# Autodesk Inventor assembly: ENSAMBLE MECANISMO DE INGRESO
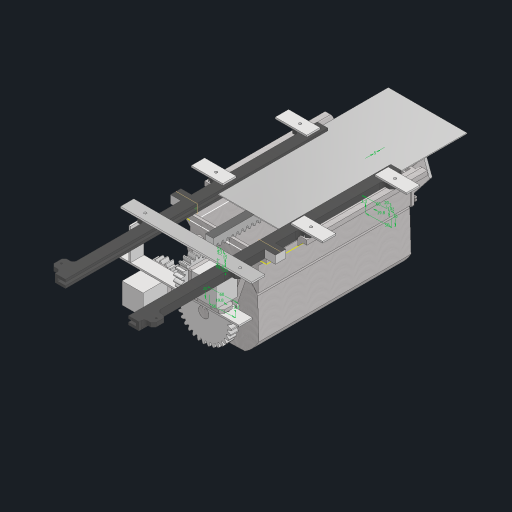
[picture p0: Inventor's stored thumbnail of the model, 512x512]
Saved by Autodesk Inventor 2024.3 (Build 283343000, 343)
## iProperties
Created: 2024-06-13
Part Number: ENSAMBLE MECANISMO DE INGRESO
Document SubType Name: Assembly
Designer: Jhuliams
Author: Jhuliams
## Documents named in this file (25)
- C:\Users\Niler\OneDrive\Escritorio\RECICLADOR\RECICLADOR_MODELO_3D\MECANISMO DE COMPACTADO\ENSAMBLE MECANISMO DE INGRESO.iam
- C:\Users\Niler\OneDrive\Escritorio\RECICLADOR\RECICLADOR_MODELO_3D\MECANISMO DE COMPACTADO\PINON DE TAPA PRINCIPAL.ipt
- C:\Users\Niler\OneDrive\Escritorio\RECICLADOR\RECICLADOR_MODELO_3D\MECANISMO DE COMPACTADO\TAPA PRICIPAL CON CREMALLERA.ipt
- C:\Users\Niler\OneDrive\Escritorio\RECICLADOR\RECICLADOR_MODELO_3D\MECANISMO DE COMPACTADO\GUIA DE TAPA PRINCIPAL.ipt
- C:\Users\Niler\OneDrive\Escritorio\RECICLADOR\RECICLADOR_MODELO_3D\MECANISMO DE COMPACTADO\NEMA 17 PARA TAPA PRINCIPAL.ipt
- C:\Users\Niler\OneDrive\Escritorio\RECICLADOR\RECICLADOR_MODELO_3D\MECANISMO DE COMPACTADO\PLETINA PARA CARA INCLINADA.ipt
- C:\Users\Niler\OneDrive\Escritorio\RECICLADOR\RECICLADOR_MODELO_3D\MECANISMO DE COMPACTADO\PLETINA PARA CARA INCLINADA_2.ipt
- C:\Users\Niler\OneDrive\Escritorio\RECICLADOR\RECICLADOR_MODELO_3D\MECANISMO DE COMPACTADO\ACOPLE_NEMA_PUERTA.ipt
- C:\Users\Niler\OneDrive\Escritorio\RECICLADOR\RECICLADOR_MODELO_3D\MECANISMO DE COMPACTADO\TOBOGAN_BASURA.ipt
- C:\Users\Niler\OneDrive\Escritorio\RECICLADOR\RECICLADOR_MODELO_3D\MECANISMO DE COMPACTADO\COMPUERTA_ALUMINIO.ipt
- C:\Users\Niler\OneDrive\Escritorio\RECICLADOR\RECICLADOR_MODELO_3D\MECANISMO DE COMPACTADO\PUERTA_ACOPLE_ENTRADA_v2.ipt
- C:\Users\Niler\OneDrive\Escritorio\RECICLADOR\RECICLADOR_MODELO_3D\MECANISMO DE COMPACTADO\CAJA_V2.ipt
- C:\Users\Niler\OneDrive\Escritorio\RECICLADOR\RECICLADOR_MODELO_3D\MECANISMO DE COMPACTADO\GIRO_1.ipt
- C:\Users\Niler\OneDrive\Escritorio\RECICLADOR\RECICLADOR_MODELO_3D\MECANISMO DE COMPACTADO\GIRO_2.ipt
- C:\Users\Niler\OneDrive\Escritorio\RECICLADOR\RECICLADOR_MODELO_3D\MECANISMO DE COMPACTADO\SOPORTE_RODAMIENTO.ipt
- C:\Users\Niler\OneDrive\Escritorio\RECICLADOR\RECICLADOR_MODELO_3D\MECANISMO DE COMPACTADO\ACOPLE_NEMA_PUERTA_V2.ipt
- C:\Users\Niler\OneDrive\Escritorio\RECICLADOR\RECICLADOR_MODELO_3D\MECANISMO DE COMPACTADO\ENGRANAJE CONDUCTOR DE CAJA.ipt
- C:\Users\Niler\OneDrive\Escritorio\RECICLADOR\RECICLADOR_MODELO_3D\MECANISMO DE COMPACTADO\ENGRANE MOTRIZ DE CAJA.ipt
- C:\Users\Niler\OneDrive\Escritorio\RECICLADOR\RECICLADOR_MODELO_3D\MECANISMO DE COMPACTADO\MUESCA_DETECCION_CERO.ipt
- C:\Users\Niler\OneDrive\Escritorio\RECICLADOR\RECICLADOR_MODELO_3D\VERSION_3_COMPLETA\CAMARA.ipt
- C:\Users\Niler\OneDrive\Escritorio\RECICLADOR\RECICLADOR_MODELO_3D\VERSION_3_COMPLETA\SOPORTE_CAMARA_2.ipt
- C:\Users\Niler\OneDrive\Escritorio\RECICLADOR\RECICLADOR_MODELO_3D\VERSION_3_COMPLETA\FIN_DE_CARRERA.ipt
- C:\Users\Niler\OneDrive\Escritorio\RECICLADOR\RECICLADOR_MODELO_3D\VERSION_3_COMPLETA\SOPORTE_FIN_CARRERA_INGRESO.ipt
- C:\Users\Niler\OneDrive\Escritorio\RECICLADOR\RECICLADOR_MODELO_3D\VERSION_3_COMPLETA\CIRCULAR_FIN_DE_CARRERA.ipt
- C:\Users\Niler\OneDrive\Escritorio\RECICLADOR\RECICLADOR_MODELO_3D\VERSION_3_COMPLETA\TAPA_CAMARA_2.ipt
## Components (34 placed, 24 different names)
1. PINON DE TAPA PRINCIPAL:1 — Mate:7, Mate:8, Mate:29, Flush:20, Rotation/Translation:1
2. NEMA 17 PARA TAPA PRINCIPAL:1 — Mate:7, Mate:8, Mate:30, Mate:31, Mate:32, Angle:1
3. PLETINA PARA CARA INCLINADA:1 — Flush:16, Flush:17, Mate:12, Mate:13, Mate:14, Mate:16, Mate:24, Mate:30, Mate:33, Flush:21
4. PLETINA PARA CARA INCLINADA_2:1 — Flush:16, Mate:18, Mate:23, Flush:19
5. PLETINA PARA CARA INCLINADA_2:2 — Flush:17, Mate:19, Mate:20, Flush:18
6. GUIA DE TAPA PRINCIPAL:3 — Mate:14, Mate:16, Mate:18, Mate:23, Mate:26, Mate:28, Angle:2, Symmetry:1
7. GUIA DE TAPA PRINCIPAL:4 — Mate:13, Mate:19, Mate:20, Mate:24, Mate:25, Mate:27, Angle:3, Mate:42, Symmetry:1
8. TAPA PRICIPAL CON CREMALLERA:1 — Mate:29, Flush:20, Rotation/Translation:1, Mate:38, Angle:3, Mate:44, Mate:45, Mate:89
9. PLETINA PARA CARA INCLINADA_2:3 — Mate:25, Flush:18, Mate:27, Mate:37, Mate:41
10. PLETINA PARA CARA INCLINADA_2:4 — Mate:26, Flush:19, Mate:28, Mate:36, Mate:40
11. ACOPLE_NEMA_PUERTA:1 — Mate:31, Mate:32, Angle:1, Angle:2, Mate:39
12. PLETINA PARA CARA INCLINADA_2:5 — Mate:33, Flush:21, Mate:34, Flush:22
13. PLETINA PARA CARA INCLINADA:2 — Mate:34, Flush:22, Mate:35, Flush:23, Mate:39, Mate:57, Flush:26
14. PLETINA PARA CARA INCLINADA_2:6 — Mate:35, Flush:23
15. TOBOGAN_BASURA:1 — Mate:36, Mate:37
16. COMPUERTA_ALUMINIO:1 — Mate:38, Mate:44, Mate:89
17. PUERTA_ACOPLE_ENTRADA_v2:1 — Mate:40, Mate:41, Mate:42, Flush:24, Mate:43, Mate:51, Mate:52, Mate:53, Mate:55, Mate:56, Mate:79, Mate:80, Mate:81
18. CAJA_V2:1 — Flush:24, Mate:43, Mate:46, Mate:48, Mate:49, Mate:50, Mate:54, Mate:66, Mate:67, Mate:68, Mate:69
19. GIRO_1:1 — Mate:46, Mate:48, Mate:61, Flush:28, Mate:69
20. GIRO_2:1 — Mate:49, Mate:50, Mate:85, Mate:86, Mate:87
21. SOPORTE_RODAMIENTO:1 — Mate:51, Mate:52, Mate:53, Mate:73, Mate:74, Mate:75
22. SOPORTE_RODAMIENTO:2 — Mate:54, Mate:55, Mate:56
23. ACOPLE_NEMA_PUERTA_V2:1 — Mate:57, Flush:26, Mate:59, Flush:27, Mate:60
24. ENGRANAJE CONDUCTOR DE CAJA:1 — Mate:61, Flush:28
25. ENGRANE MOTRIZ DE CAJA:1 — Mate:62
26. NEMA 17 PARA TAPA PRINCIPAL:2 — Mate:59, Flush:27, Mate:60, Mate:62
27. MUESCA_DETECCION_CERO:1 — Mate:66, Mate:67, Mate:68
28. SOPORTE_CAMARA_2:1 — Mate:70, Mate:73, Mate:74, Mate:75, Mate:76, Mate:77, Mate:78, Flush:29, Mate:88
29. CAMARA:1 — Mate:70
30. FIN_DE_CARRERA:1 — Mate:76, Mate:77, Mate:78
31. SOPORTE_FIN_CARRERA_INGRESO:1 — Mate:79, Mate:80, Mate:81, Mate:82, Mate:83, Mate:84
32. FIN_DE_CARRERA:2 — Mate:82, Mate:83, Mate:84
33. CIRCULAR_FIN_DE_CARRERA:1 — Mate:85, Mate:86, Mate:87
34. TAPA_CAMARA_2:1 — Flush:29, Mate:88
## Relationships (91: Mate 70, Flush 15, Angle 3, RelateRotateTranslate 1, Symmetry 1, RelateRotation 1)
- Flush:4 (27 mm)
- Mate:7: PINON DE TAPA PRINCIPAL:1 ↔ NEMA 17 PARA TAPA PRINCIPAL:1
- Mate:8 (10 mm): PINON DE TAPA PRINCIPAL:1 ↔ NEMA 17 PARA TAPA PRINCIPAL:1
- Flush:16: PLETINA PARA CARA INCLINADA:1 ↔ PLETINA PARA CARA INCLINADA_2:1
- Flush:17: PLETINA PARA CARA INCLINADA:1 ↔ PLETINA PARA CARA INCLINADA_2:2
- Mate:12: PLETINA PARA CARA INCLINADA:1
- Mate:13: PLETINA PARA CARA INCLINADA:1 ↔ GUIA DE TAPA PRINCIPAL:4
- Mate:14: PLETINA PARA CARA INCLINADA:1 ↔ GUIA DE TAPA PRINCIPAL:3
- Mate:16: PLETINA PARA CARA INCLINADA:1 ↔ GUIA DE TAPA PRINCIPAL:3
- Mate:18: PLETINA PARA CARA INCLINADA_2:1 ↔ GUIA DE TAPA PRINCIPAL:3
- Mate:19: PLETINA PARA CARA INCLINADA_2:2 ↔ GUIA DE TAPA PRINCIPAL:4
- Mate:20: PLETINA PARA CARA INCLINADA_2:2 ↔ GUIA DE TAPA PRINCIPAL:4
- Mate:23: PLETINA PARA CARA INCLINADA_2:1 ↔ GUIA DE TAPA PRINCIPAL:3
- Mate:24: PLETINA PARA CARA INCLINADA:1 ↔ GUIA DE TAPA PRINCIPAL:4
- Mate:25: GUIA DE TAPA PRINCIPAL:4 ↔ PLETINA PARA CARA INCLINADA_2:3
- Flush:18: PLETINA PARA CARA INCLINADA_2:2 ↔ PLETINA PARA CARA INCLINADA_2:3
- Mate:26: GUIA DE TAPA PRINCIPAL:3 ↔ PLETINA PARA CARA INCLINADA_2:4
- Flush:19: PLETINA PARA CARA INCLINADA_2:1 ↔ PLETINA PARA CARA INCLINADA_2:4
- Mate:27: GUIA DE TAPA PRINCIPAL:4 ↔ PLETINA PARA CARA INCLINADA_2:3
- Mate:28: GUIA DE TAPA PRINCIPAL:3 ↔ PLETINA PARA CARA INCLINADA_2:4
- Mate:29 (30.4 mm): PINON DE TAPA PRINCIPAL:1 ↔ TAPA PRICIPAL CON CREMALLERA:1
- Flush:20: PINON DE TAPA PRINCIPAL:1 ↔ TAPA PRICIPAL CON CREMALLERA:1
- Mate:30: NEMA 17 PARA TAPA PRINCIPAL:1 ↔ PLETINA PARA CARA INCLINADA:1
- Rotation/Translation:1 [RelateRotateTranslate] (169 mm): PINON DE TAPA PRINCIPAL:1 ↔ TAPA PRICIPAL CON CREMALLERA:1
- Mate:31: NEMA 17 PARA TAPA PRINCIPAL:1 ↔ ACOPLE_NEMA_PUERTA:1
- Mate:32: NEMA 17 PARA TAPA PRINCIPAL:1 ↔ ACOPLE_NEMA_PUERTA:1
- Angle:1 (0 deg): NEMA 17 PARA TAPA PRINCIPAL:1 ↔ ACOPLE_NEMA_PUERTA:1
- Angle:2 (0 deg): GUIA DE TAPA PRINCIPAL:3 ↔ ACOPLE_NEMA_PUERTA:1
- Mate:33 (20 mm): PLETINA PARA CARA INCLINADA:1 ↔ PLETINA PARA CARA INCLINADA_2:5
- Flush:21: PLETINA PARA CARA INCLINADA:1 ↔ PLETINA PARA CARA INCLINADA_2:5
- Mate:34: PLETINA PARA CARA INCLINADA_2:5 ↔ PLETINA PARA CARA INCLINADA:2
- Flush:22: PLETINA PARA CARA INCLINADA_2:5 ↔ PLETINA PARA CARA INCLINADA:2
- Mate:35: PLETINA PARA CARA INCLINADA:2 ↔ PLETINA PARA CARA INCLINADA_2:6
- Flush:23: PLETINA PARA CARA INCLINADA:2 ↔ PLETINA PARA CARA INCLINADA_2:6
- Mate:36: PLETINA PARA CARA INCLINADA_2:4 ↔ TOBOGAN_BASURA:1
- Mate:37: PLETINA PARA CARA INCLINADA_2:3 ↔ TOBOGAN_BASURA:1
- Mate:38: TAPA PRICIPAL CON CREMALLERA:1 ↔ COMPUERTA_ALUMINIO:1
- Mate:39: ACOPLE_NEMA_PUERTA:1 ↔ PLETINA PARA CARA INCLINADA:2
- Angle:3 (0 deg): GUIA DE TAPA PRINCIPAL:4 ↔ TAPA PRICIPAL CON CREMALLERA:1
- Mate:40: PLETINA PARA CARA INCLINADA_2:4 ↔ PUERTA_ACOPLE_ENTRADA_v2:1
- Mate:41: PLETINA PARA CARA INCLINADA_2:3 ↔ PUERTA_ACOPLE_ENTRADA_v2:1
- Mate:42: GUIA DE TAPA PRINCIPAL:4 ↔ PUERTA_ACOPLE_ENTRADA_v2:1
- Flush:24: PUERTA_ACOPLE_ENTRADA_v2:1 ↔ CAJA_V2:1
- Mate:43: PUERTA_ACOPLE_ENTRADA_v2:1 ↔ CAJA_V2:1
- Mate:44: TAPA PRICIPAL CON CREMALLERA:1 ↔ COMPUERTA_ALUMINIO:1
- Symmetry:1: GUIA DE TAPA PRINCIPAL:3 ↔ GUIA DE TAPA PRINCIPAL:4
- Mate:45: TAPA PRICIPAL CON CREMALLERA:1
- Mate:46: CAJA_V2:1 ↔ GIRO_1:1
- Mate:48: CAJA_V2:1 ↔ GIRO_1:1
- Mate:49: CAJA_V2:1 ↔ GIRO_2:1
- Mate:50: CAJA_V2:1 ↔ GIRO_2:1
- Mate:51: PUERTA_ACOPLE_ENTRADA_v2:1 ↔ SOPORTE_RODAMIENTO:1
- Mate:52: PUERTA_ACOPLE_ENTRADA_v2:1 ↔ SOPORTE_RODAMIENTO:1
- Mate:53: PUERTA_ACOPLE_ENTRADA_v2:1 ↔ SOPORTE_RODAMIENTO:1
- Mate:54: CAJA_V2:1 ↔ SOPORTE_RODAMIENTO:2
- Mate:55: PUERTA_ACOPLE_ENTRADA_v2:1 ↔ SOPORTE_RODAMIENTO:2
- Mate:56: PUERTA_ACOPLE_ENTRADA_v2:1 ↔ SOPORTE_RODAMIENTO:2
- Mate:57: PLETINA PARA CARA INCLINADA:2 ↔ ACOPLE_NEMA_PUERTA_V2:1
- [Flush]: ENGRANAJE CONDUCTOR DE CAJA:1 ↔ ENGRANE MOTRIZ DE CAJA:1
- [Mate] (79.5 mm): ENGRANAJE CONDUCTOR DE CAJA:1 ↔ ENGRANE MOTRIZ DE CAJA:1
- [RelateRotation] (1.65 ul): ENGRANAJE CONDUCTOR DE CAJA:1 ↔ ENGRANE MOTRIZ DE CAJA:1
- Flush:26 (-5 mm): PLETINA PARA CARA INCLINADA:2 ↔ ACOPLE_NEMA_PUERTA_V2:1
- Mate:59: ACOPLE_NEMA_PUERTA_V2:1 ↔ NEMA 17 PARA TAPA PRINCIPAL:2
- Flush:27: ACOPLE_NEMA_PUERTA_V2:1 ↔ NEMA 17 PARA TAPA PRINCIPAL:2
- Mate:60: ACOPLE_NEMA_PUERTA_V2:1 ↔ NEMA 17 PARA TAPA PRINCIPAL:2
- Mate:61: GIRO_1:1 ↔ ENGRANAJE CONDUCTOR DE CAJA:1
- Mate:62: ENGRANE MOTRIZ DE CAJA:1 ↔ NEMA 17 PARA TAPA PRINCIPAL:2
- Flush:28: GIRO_1:1 ↔ ENGRANAJE CONDUCTOR DE CAJA:1
- Mate:66: CAJA_V2:1 ↔ MUESCA_DETECCION_CERO:1
- Mate:67: CAJA_V2:1 ↔ MUESCA_DETECCION_CERO:1
- Mate:68: CAJA_V2:1 ↔ MUESCA_DETECCION_CERO:1
- Mate:69: CAJA_V2:1 ↔ GIRO_1:1
- Mate:70: SOPORTE_CAMARA_2:1 ↔ CAMARA:1
- Mate:73: SOPORTE_RODAMIENTO:1 ↔ SOPORTE_CAMARA_2:1
- Mate:74: SOPORTE_RODAMIENTO:1 ↔ SOPORTE_CAMARA_2:1
- Mate:75: SOPORTE_RODAMIENTO:1 ↔ SOPORTE_CAMARA_2:1
- Mate:76: SOPORTE_CAMARA_2:1 ↔ FIN_DE_CARRERA:1
- Mate:77: SOPORTE_CAMARA_2:1 ↔ FIN_DE_CARRERA:1
- Mate:78: SOPORTE_CAMARA_2:1 ↔ FIN_DE_CARRERA:1
- Mate:79: PUERTA_ACOPLE_ENTRADA_v2:1 ↔ SOPORTE_FIN_CARRERA_INGRESO:1
- Mate:80: PUERTA_ACOPLE_ENTRADA_v2:1 ↔ SOPORTE_FIN_CARRERA_INGRESO:1
- Mate:81: PUERTA_ACOPLE_ENTRADA_v2:1 ↔ SOPORTE_FIN_CARRERA_INGRESO:1
- Mate:82: SOPORTE_FIN_CARRERA_INGRESO:1 ↔ FIN_DE_CARRERA:2
- Mate:83: SOPORTE_FIN_CARRERA_INGRESO:1 ↔ FIN_DE_CARRERA:2
- Mate:84: SOPORTE_FIN_CARRERA_INGRESO:1 ↔ FIN_DE_CARRERA:2
- Mate:85: GIRO_2:1 ↔ CIRCULAR_FIN_DE_CARRERA:1
- Mate:86: GIRO_2:1 ↔ CIRCULAR_FIN_DE_CARRERA:1
- Mate:87: GIRO_2:1 ↔ CIRCULAR_FIN_DE_CARRERA:1
- Flush:29: SOPORTE_CAMARA_2:1 ↔ TAPA_CAMARA_2:1
- Mate:88: SOPORTE_CAMARA_2:1 ↔ TAPA_CAMARA_2:1
- Mate:89: TAPA PRICIPAL CON CREMALLERA:1 ↔ COMPUERTA_ALUMINIO:1
